# Autodesk Inventor assembly: bumper
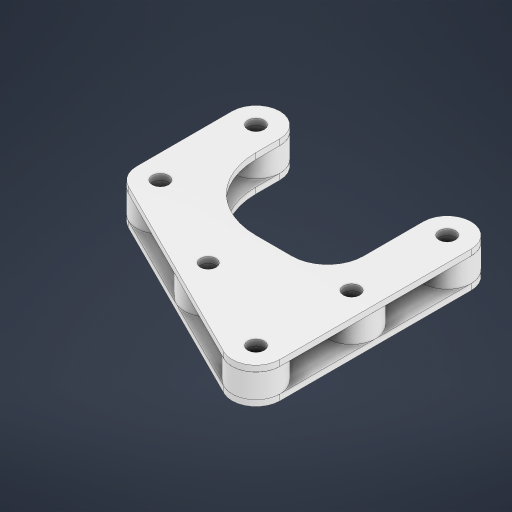
[picture p0: Inventor's stored thumbnail of the model, 512x512]
Saved by Autodesk Inventor 2024 (Build 280153000, 153)
## iProperties
Created: 2024-01-15
Part Number: bumper
Document SubType Name: Assembly
Designer: avere
Author: avere
## Documents named in this file (4)
- C:\Users\avere\Documents\rbp_cad\zoomba_v0.3\chassis\drivebay\bumper.iam
- C:\Users\avere\Documents\rbp_cad\zoomba_v0.3\chassis\drivebay\custom_parts\gusset.ipt
- C:\Users\avere\Documents\rbp_cad\VEX-CAD-Inventor-1.41\Motion\Spacers\Spacer Nylon .500 OD\NSpacer White .500 OD x .250.ipt
- C:\Users\avere\Documents\rbp_cad\VEX-CAD-Inventor-1.41\Motion\Spacers\Spacer Nylon .500 OD.ipt
## Components (8 placed, 2 different names)
1. gusset:1 — Insert:1, Insert:2, Insert:5, Insert:7, Insert:9
2. gusset:2 — Insert:3, Insert:4, Insert:6, Insert:8, Insert:10
3. NSpacer White .500 OD x .250:1 — Insert:2, Insert:4
4. NSpacer White .500 OD x .250:2 — Insert:1, Insert:3
5. NSpacer White .500 OD x .250:3 — Insert:5, Insert:6
6. NSpacer White .500 OD x .250:4 — Insert:7, Insert:8
7. NSpacer White .500 OD x .250:5 — Insert:9
8. NSpacer White .500 OD x .250:6 — Insert:10
## Relationships (10: Insert 10)
- Insert:1: gusset:1 ↔ NSpacer White .500 OD x .250:2
- Insert:2: gusset:1 ↔ NSpacer White .500 OD x .250:1
- Insert:3: gusset:2 ↔ NSpacer White .500 OD x .250:2
- Insert:4: gusset:2 ↔ NSpacer White .500 OD x .250:1
- Insert:5: gusset:1 ↔ NSpacer White .500 OD x .250:3
- Insert:6: gusset:2 ↔ NSpacer White .500 OD x .250:3
- Insert:7: gusset:1 ↔ NSpacer White .500 OD x .250:4
- Insert:8: gusset:2 ↔ NSpacer White .500 OD x .250:4
- Insert:9: gusset:1 ↔ NSpacer White .500 OD x .250:5
- Insert:10: gusset:2 ↔ NSpacer White .500 OD x .250:6
